# Autodesk Inventor assembly: Cuvette
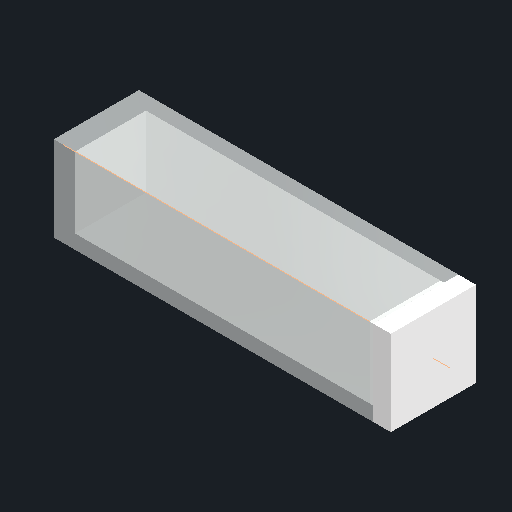
[picture p0: Inventor's stored thumbnail of the model, 512x512]
Saved by Autodesk Inventor 2024.1 (Build 281209000, 209)
## iProperties
Created: 2024-08-12
Part Number: Cuvette
Document SubType Name: Assembly
Designer: Tim Jäger
Author: Tim Jäger
## Documents named in this file (3)
- D:\Users\Tim\VUB\Master_Embedded\Master_Thesis\Files3D\Cuvette.iam
- D:\Users\Tim\VUB\Master_Embedded\Master_Thesis\Files3D\Cuvette.ipt
- D:\Users\Tim\VUB\Master_Embedded\Master_Thesis\Files3D\Cuvette_Lid.ipt
## Components (2 placed, 2 different names)
1. Cuvette:1 — Mate:1, Mate:2, Mate:3
2. Cuvette_Lid:1 — Mate:1, Mate:2, Mate:3
## Relationships (3: Mate 3)
- Mate:1: Cuvette:1 ↔ Cuvette_Lid:1
- Mate:2: Cuvette:1 ↔ Cuvette_Lid:1
- Mate:3: Cuvette:1 ↔ Cuvette_Lid:1
